# Autodesk Inventor assembly: Shooter_assembly
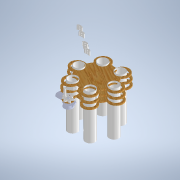
[picture p0: Inventor's stored thumbnail of the model, 180x180]
Saved by Autodesk Inventor 2020.2 (Build 242310000, 310)
## iProperties
Created: 2019-11-06
Part Number: Shooter_assembly
Document SubType Name: Assembly
Designer: Paul Lefeuvre
Mass: 3189.14 g
Surface Area: 13283.7 cm^2
Volume: 3064.78 cm^3
Density: 1.04058 g/cm^3
Author: Paul Lefeuvre
## Documents named in this file (9)
- C:\Users\Paul Lefeuvre\Documents\Inventor\T-Shirt_Cannon\Shooter_assembly.iam
- C:\Users\Paul Lefeuvre\Documents\Inventor\T-Shirt_Cannon\AmmoHolder.ipt
- C:\Users\Paul Lefeuvre\Documents\Inventor\T-Shirt_Cannon\GenevaHolder.ipt
- C:\Users\Paul Lefeuvre\Documents\Inventor\T-Shirt_Cannon\PVC_pipe.ipt
- C:\Users\Paul Lefeuvre\Documents\Inventor\T-Shirt_Cannon\am-2235a Snow Blower Motor With Hex Shaft.ipt
- C:\Users\Paul Lefeuvre\Documents\Inventor\T-Shirt_Cannon\GenevaDrive3.ipt
- C:\Users\Paul Lefeuvre\Documents\Inventor\T-Shirt_Cannon\GenevaDrive2.ipt
- C:\Users\Paul Lefeuvre\Documents\Inventor\T-Shirt_Cannon\GenevaPin.ipt
- C:\Users\Paul Lefeuvre\Documents\Inventor\T-Shirt_Cannon\PipeHolder.ipt
## Components (25 placed, 8 different names)
1. AmmoHolder:1 — Insert:7, Insert:13, Insert:20, Insert:21, Insert:22, Insert:23, Insert:24, Insert:25, Insert:26, Insert:27, Insert:28, Mate:1, Insert:29, Insert:30
2. GenevaHolder:1 — Insert:6, Insert:14, Insert:15, Insert:16, Insert:17, Insert:18, Insert:19
3. PVC_pipe:1 — Insert:7, Insert:8, Insert:18
4. PVC_pipe:2 — Insert:12, Insert:13, Insert:19
5. PVC_pipe:3 — Insert:6, Insert:17
6. PVC_pipe:4 — Insert:15
7. PVC_pipe:5 — Insert:14
8. PVC_pipe:6 — Insert:16
9. am-2235a Snow Blower Motor With Hex Shaft:1 — Rotational:10
10. AmmoHolder:2 — Insert:8, Insert:12
11. GenevaDrive3:1 — Rigid:13, Rigid:14
12. GenevaDrive2:1 — Rigid:13, Rotational:10
13. GenevaPin:1 — Rigid:14
14. PipeHolder:1
15. PipeHolder:2
16. PipeHolder:3 — Insert:22, Insert:23
17. PipeHolder:4 — Insert:24, Insert:25
18. PipeHolder:5
19. PipeHolder:6 — Insert:29, Insert:30
20. PipeHolder:7
21. PipeHolder:8
22. PipeHolder:9 — Insert:28, Mate:1
23. PipeHolder:10
24. PipeHolder:11 — Insert:20, Insert:21
25. PipeHolder:12 — Insert:26, Insert:27
## Relationships (26: Insert 22, WeldJoint 2, RevoluteJoint 1, Mate 1)
- Rigid:13 [WeldJoint]: GenevaDrive3:1 ↔ GenevaDrive2:1
- Rotational:10 [RevoluteJoint] (10 mm): am-2235a Snow Blower Motor With Hex Shaft:1 ↔ GenevaDrive2:1
- Rigid:14 [WeldJoint]: GenevaDrive3:1 ↔ GenevaPin:1
- Insert:6 (-10 mm): GenevaHolder:1 ↔ PVC_pipe:3
- Insert:7 (-50 mm): AmmoHolder:1 ↔ PVC_pipe:1
- Insert:8 (-90 mm): PVC_pipe:1 ↔ AmmoHolder:2
- Insert:12 (-90 mm): PVC_pipe:2 ↔ AmmoHolder:2
- Insert:13 (-50 mm): AmmoHolder:1 ↔ PVC_pipe:2
- Insert:14 (-10 mm): GenevaHolder:1 ↔ PVC_pipe:5
- Insert:15 (-10 mm): GenevaHolder:1 ↔ PVC_pipe:4
- Insert:16 (-10 mm): GenevaHolder:1 ↔ PVC_pipe:6
- Insert:17 (-10 mm): GenevaHolder:1 ↔ PVC_pipe:3
- Insert:18 (-10 mm): GenevaHolder:1 ↔ PVC_pipe:1
- Insert:19 (-10 mm): GenevaHolder:1 ↔ PVC_pipe:2
- Insert:20 (0.3 mm): AmmoHolder:1 ↔ PipeHolder:11
- Insert:21 (0.3 mm): AmmoHolder:1 ↔ PipeHolder:11
- Insert:22 (0.3 mm): AmmoHolder:1 ↔ PipeHolder:3
- Insert:23 (0.3 mm): AmmoHolder:1 ↔ PipeHolder:3
- Insert:24 (0.3 mm): AmmoHolder:1 ↔ PipeHolder:4
- Insert:25 (0.3 mm): AmmoHolder:1 ↔ PipeHolder:4
- Insert:26 (0.3 mm): AmmoHolder:1 ↔ PipeHolder:12
- Insert:27 (0.3 mm): AmmoHolder:1 ↔ PipeHolder:12
- Insert:28 (0.3 mm): AmmoHolder:1 ↔ PipeHolder:9
- Mate:1 (0.3 mm): AmmoHolder:1 ↔ PipeHolder:9
- Insert:29 (0.3 mm): AmmoHolder:1 ↔ PipeHolder:6
- Insert:30 (0.3 mm): AmmoHolder:1 ↔ PipeHolder:6
## Named parameters: sa_0 = 45000
note: some values were not read from the file. Shown as the stored number, unit unknown: "sa_0".
